# Autodesk Inventor assembly: КВ33.044.300 -  Сборка мотора Makeblock с крепление
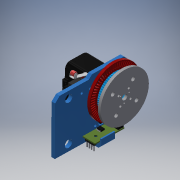
[picture p0: Inventor's stored thumbnail of the model, 180x180]
Saved by Autodesk Inventor 2019 (Build 230136000, 136)
## iProperties
Created: 2019-07-17
Part Number: КВ33.044.300 -  Сборка мотора Makeblock с крепление
Material: Типовые
Document SubType Name: Assembly
Designer: Петров Иван
Author: Петров Иван
## Documents named in this file (9)
- E:\IVAN\Kvantoriada2019\optimal_gripper\hardware\КВ33.044.500 -  Сборка сервомотора Dynamixel с крепление.iam
- E:\IVAN\Kvantoriada2019\optimal_gripper\hardware\КВ33.044.501 - Деражатель мотора.ipt
- E:\IVAN\Kvantoriada2019\optimal_gripper\hardware\Стандартные изделия\Проставка 4 мм.ipt
- E:\IVAN\Kvantoriada2019\optimal_gripper\hardware\Стандартные изделия\Колесо оптического датчика.ipt
- E:\IVAN\Kvantoriada2019\optimal_gripper\hardware\Стандартные изделия\Шкив большой Makeblock.ipt
- E:\IVAN\Kvantoriada2019\optimal_gripper\hardware\Стандартные изделия\Сервомотор Dynamixel AX-12A\AX-12.iam
- E:\IVAN\Kvantoriada2019\optimal_gripper\hardware\Стандартные изделия\Боковина шкива.ipt
- E:\IVAN\Kvantoriada2019\optimal_gripper\hardware\Стандартные изделия\Датчик оптический с измененными контактами.ipt
- E:\IVAN\Kvantoriada2019\optimal_gripper\hardware\Стандартные изделия\Концевик механический.ipt
## Components (8 placed, 8 different names)
1. КВ33.044.501 - Деражатель мотора:1 — Совмещение:1, Совмещение:2, Совмещение:23, Совмещение:19, Заподлицо:2, Совмещение:20, Совмещение:21, Совмещение:22, Совмещение:24, Совмещение:25, Совмещение:26
2. Проставка 4 мм:1 — Совмещение:1, Совмещение:2, Совмещение:10, Совмещение:12
3. Шкив большой Makeblock:1 — Совмещение:13, Совмещение:14, Совмещение:15, Совмещение:16, Совмещение:17, Совмещение:18
4. AX-12:1 [sub-assembly] — Совмещение:24, Совмещение:25, Совмещение:26
5. Колесо оптического датчика:1 — Совмещение:10, Совмещение:12, Совмещение:13, Совмещение:14, Совмещение:15
6. Боковина шкива:1 — Совмещение:16, Совмещение:17, Совмещение:18
7. Датчик оптический с измененными контактами:1 — Совмещение:23, Совмещение:19, Заподлицо:2
8. Концевик механический:1 — Совмещение:20, Совмещение:21, Совмещение:22
## Relationships (19: Mate 18, Flush 1)
- Совмещение:1 [Mate]: КВ33.044.501 - Деражатель мотора:1 ↔ Проставка 4 мм:1
- Совмещение:2 [Mate]: КВ33.044.501 - Деражатель мотора:1 ↔ Проставка 4 мм:1
- Совмещение:10 [Mate]: Проставка 4 мм:1 ↔ Колесо оптического датчика:1
- Совмещение:12 [Mate]: Проставка 4 мм:1 ↔ Колесо оптического датчика:1
- Совмещение:13 [Mate]: Шкив большой Makeblock:1 ↔ Колесо оптического датчика:1
- Совмещение:14 [Mate]: Шкив большой Makeblock:1 ↔ Колесо оптического датчика:1
- Совмещение:15 [Mate]: Шкив большой Makeblock:1 ↔ Колесо оптического датчика:1
- Совмещение:16 [Mate]: Шкив большой Makeblock:1 ↔ Боковина шкива:1
- Совмещение:17 [Mate]: Шкив большой Makeblock:1 ↔ Боковина шкива:1
- Совмещение:18 [Mate]: Шкив большой Makeblock:1 ↔ Боковина шкива:1
- Совмещение:23 [Mate]: КВ33.044.501 - Деражатель мотора:1 ↔ Датчик оптический с измененными контактами:1
- Совмещение:19 [Mate]: КВ33.044.501 - Деражатель мотора:1 ↔ Датчик оптический с измененными контактами:1
- Заподлицо:2 [Flush] (13 mm): КВ33.044.501 - Деражатель мотора:1 ↔ Датчик оптический с измененными контактами:1
- Совмещение:20 [Mate]: КВ33.044.501 - Деражатель мотора:1 ↔ Концевик механический:1
- Совмещение:21 [Mate]: КВ33.044.501 - Деражатель мотора:1 ↔ Концевик механический:1
- Совмещение:22 [Mate]: КВ33.044.501 - Деражатель мотора:1 ↔ Концевик механический:1
- Совмещение:24 [Mate]: КВ33.044.501 - Деражатель мотора:1 ↔ AX-12:1
- Совмещение:25 [Mate]: КВ33.044.501 - Деражатель мотора:1 ↔ AX-12:1
- Совмещение:26 [Mate]: КВ33.044.501 - Деражатель мотора:1 ↔ AX-12:1
